# Autodesk Inventor assembly: X-axis Motor Holder assy
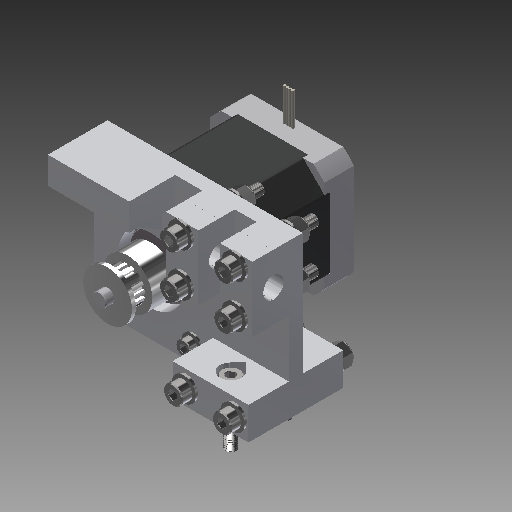
[picture p0: Inventor's stored thumbnail of the model, 512x512]
Saved by Autodesk Inventor 2018 (Build 220112000, 112)
## iProperties
Created: 2017-10-03
Part Number: X-axis Motor Holder assy
Document SubType Name: Assembly
Designer: Gabriel Smolnycki
Author: Gabriel Smolnycki
## Documents named in this file (13)
- E:\planb\mechanics\V1INV\Subassemblies\X-axis Motor Holder assy.iam
- E:\planb\mechanics\V1INV\X-axis\X-axis Motor Holder.ipt
- E:\planb\mechanics\V1INV\Electronics\ST4118L1804-B.ipt
- E:\planb\mechanics\V1INV\Hardware\M3 SS Washer.ipt
- E:\planb\mechanics\V1INV\Hardware\M3x10 SS SHCS.ipt
- E:\planb\mechanics\V1INV\Hardware\T2.5 16T Pulley.ipt
- E:\planb\mechanics\V1INV\X-axis\X-axis Holder Coupler.ipt
- E:\planb\mechanics\V1INV\Hardware\M4x20 SS SHCS.ipt
- E:\planb\mechanics\V1INV\Hardware\M4x40 SS SHCS.ipt
- E:\planb\mechanics\V1INV\Hardware\M4 SS Washer.ipt
- E:\planb\mechanics\V1INV\Hardware\M4 SS Locknut.ipt
- E:\planb\mechanics\V1INV\X-axis\X-axis Rod Holder.ipt
- E:\planb\mechanics\V1INV\Hardware\M4x30 SS SHCS.ipt
## Components (41 placed, 12 different names)
1. X-axis Motor Holder:1 — Insert:1, Insert:2, Insert:3, Insert:4, Insert:5, Insert:6, Insert:12, Insert:13, Insert:14, Insert:15, Insert:26, Insert:27, Insert:28, Insert:29, Insert:34, Insert:35, Insert:36, Insert:37, Insert:46
2. ST4118L1804-B:1 — Insert:1, Insert:2
3. M3 SS Washer:1 — Insert:6, Insert:10
4. M3 SS Washer:2 — Insert:5, Insert:8
5. M3 SS Washer:3 — Insert:4, Insert:9
6. M3 SS Washer:4 — Insert:3, Insert:7
7. M3x10 SS SHCS:1 — Insert:10
8. M3x10 SS SHCS:2 — Insert:9
9. M3x10 SS SHCS:3 — Insert:8
10. M3x10 SS SHCS:4 — Insert:7
11. T2.5 16T Pulley:1 — Insert:46
12. X-axis Holder Coupler:1 — Insert:14, Insert:15, Insert:17, Insert:20, Insert:21
13. X-axis Holder Coupler:2 — Insert:12, Insert:13, Insert:16, Insert:18, Insert:19
14. M4x20 SS SHCS:1 — Insert:16
15. M4x20 SS SHCS:2 — Insert:17
16. M4x40 SS SHCS:1 — Insert:24
17. M4x40 SS SHCS:2 — Insert:25
18. M4 SS Washer:1 — Insert:20, Insert:22
19. M4 SS Washer:2 — Insert:21, Insert:23
20. M4 SS Washer:3 — Insert:19, Insert:25
21. M4 SS Washer:4 — Insert:18, Insert:24
22. M4 SS Locknut:1 — Insert:22
23. M4 SS Locknut:2 — Insert:23
24. X-axis Rod Holder:1 — Insert:28, Insert:29, Insert:31, Insert:33
25. X-axis Rod Holder:2 — Insert:26, Insert:27, Insert:30, Insert:32
26. M4 SS Washer:5 — Insert:30, Insert:42
27. M4 SS Washer:6 — Insert:33, Insert:45
28. M4 SS Washer:7 — Insert:34, Insert:38
29. M4 SS Washer:8 — Insert:35, Insert:40
30. M4 SS Washer:9 — Insert:31, Insert:43
31. M4 SS Washer:10 — Insert:32, Insert:44
32. M4 SS Washer:11 — Insert:36, Insert:39
33. M4 SS Washer:12 — Insert:37, Insert:41
34. M4 SS Locknut:3 — Insert:41
35. M4 SS Locknut:4 — Insert:40
36. M4 SS Locknut:5 — Insert:39
37. M4 SS Locknut:6 — Insert:38
38. M4x30 SS SHCS:1 — Insert:45
39. M4x30 SS SHCS:2 — Insert:44
40. M4x30 SS SHCS:3 — Insert:43
41. M4x30 SS SHCS:4 — Insert:42
## Relationships (45: Insert 45)
- Insert:1: X-axis Motor Holder:1 ↔ ST4118L1804-B:1
- Insert:2: X-axis Motor Holder:1 ↔ ST4118L1804-B:1
- Insert:3: X-axis Motor Holder:1 ↔ M3 SS Washer:4
- Insert:4: X-axis Motor Holder:1 ↔ M3 SS Washer:3
- Insert:5: X-axis Motor Holder:1 ↔ M3 SS Washer:2
- Insert:6: X-axis Motor Holder:1 ↔ M3 SS Washer:1
- Insert:7: M3 SS Washer:4 ↔ M3x10 SS SHCS:4
- Insert:8: M3 SS Washer:2 ↔ M3x10 SS SHCS:3
- Insert:9: M3 SS Washer:3 ↔ M3x10 SS SHCS:2
- Insert:10: M3 SS Washer:1 ↔ M3x10 SS SHCS:1
- Insert:12: X-axis Motor Holder:1 ↔ X-axis Holder Coupler:2
- Insert:13: X-axis Motor Holder:1 ↔ X-axis Holder Coupler:2
- Insert:14: X-axis Motor Holder:1 ↔ X-axis Holder Coupler:1
- Insert:15: X-axis Motor Holder:1 ↔ X-axis Holder Coupler:1
- Insert:16: X-axis Holder Coupler:2 ↔ M4x20 SS SHCS:1
- Insert:17: X-axis Holder Coupler:1 ↔ M4x20 SS SHCS:2
- Insert:18: X-axis Holder Coupler:2 ↔ M4 SS Washer:4
- Insert:19: X-axis Holder Coupler:2 ↔ M4 SS Washer:3
- Insert:20: X-axis Holder Coupler:1 ↔ M4 SS Washer:1
- Insert:21: X-axis Holder Coupler:1 ↔ M4 SS Washer:2
- Insert:22: M4 SS Washer:1 ↔ M4 SS Locknut:1
- Insert:23: M4 SS Washer:2 ↔ M4 SS Locknut:2
- Insert:24: M4x40 SS SHCS:1 ↔ M4 SS Washer:4
- Insert:25: M4x40 SS SHCS:2 ↔ M4 SS Washer:3
- Insert:26: X-axis Motor Holder:1 ↔ X-axis Rod Holder:2
- Insert:27: X-axis Motor Holder:1 ↔ X-axis Rod Holder:2
- Insert:28: X-axis Motor Holder:1 ↔ X-axis Rod Holder:1
- Insert:29: X-axis Motor Holder:1 ↔ X-axis Rod Holder:1
- Insert:30: X-axis Rod Holder:2 ↔ M4 SS Washer:5
- Insert:31: X-axis Rod Holder:1 ↔ M4 SS Washer:9
- Insert:32: X-axis Rod Holder:2 ↔ M4 SS Washer:10
- Insert:33: X-axis Rod Holder:1 ↔ M4 SS Washer:6
- Insert:34: X-axis Motor Holder:1 ↔ M4 SS Washer:7
- Insert:35: X-axis Motor Holder:1 ↔ M4 SS Washer:8
- Insert:36: X-axis Motor Holder:1 ↔ M4 SS Washer:11
- Insert:37: X-axis Motor Holder:1 ↔ M4 SS Washer:12
- Insert:38: M4 SS Washer:7 ↔ M4 SS Locknut:6
- Insert:39: M4 SS Washer:11 ↔ M4 SS Locknut:5
- Insert:40: M4 SS Washer:8 ↔ M4 SS Locknut:4
- Insert:41: M4 SS Washer:12 ↔ M4 SS Locknut:3
- Insert:42: M4 SS Washer:5 ↔ M4x30 SS SHCS:4
- Insert:43: M4 SS Washer:9 ↔ M4x30 SS SHCS:3
- Insert:44: M4 SS Washer:10 ↔ M4x30 SS SHCS:2
- Insert:45: M4 SS Washer:6 ↔ M4x30 SS SHCS:1
- Insert:46: X-axis Motor Holder:1 ↔ T2.5 16T Pulley:1
